# Autodesk Inventor assembly: robot
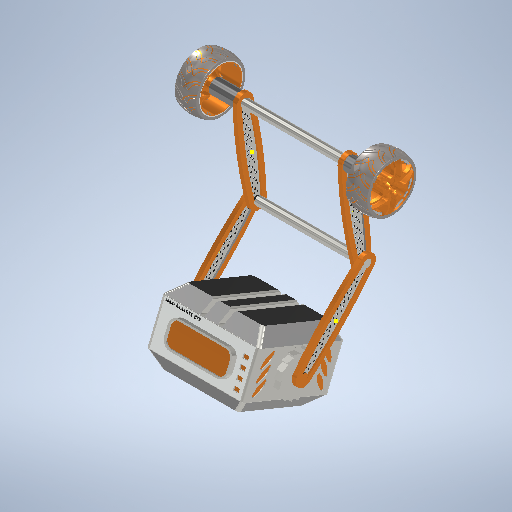
[picture p0: Inventor's stored thumbnail of the model, 512x512]
Saved by Autodesk Inventor 2025 (Build 290162000, 162)
## iProperties
Created: 2024-05-31
Part Number: robot
Document SubType Name: Assembly
Designer: bartek
Author: bartek
## Documents named in this file (6)
- C:\Users\barte\Desktop\Studia\VI semestr\Roboty mobilne\Projekt\Roboty-mobilne\robot.iam
- C:\Users\barte\Desktop\Studia\VI semestr\Roboty mobilne\Projekt\Roboty-mobilne\ipt\wheel.ipt
- C:\Users\barte\Desktop\Studia\VI semestr\Roboty mobilne\Projekt\Roboty-mobilne\ipt\engine.ipt
- C:\Users\barte\Desktop\Studia\VI semestr\Roboty mobilne\Projekt\Roboty-mobilne\ipt\link.ipt
- C:\Users\barte\Desktop\Studia\VI semestr\Roboty mobilne\Projekt\Roboty-mobilne\ipt\bolt.ipt
- C:\Users\barte\Desktop\Studia\VI semestr\Roboty mobilne\Projekt\Roboty-mobilne\ipt\body.ipt
## Components (11 placed, 5 different names)
1. wheel:1 — Rigid:1
2. wheel:2 — Rigid:2, Mate:1
3. engine:1 — Rigid:2, Mate:1, Rotational:2, Rotational:4
4. engine:2 — Rigid:1, Rotational:1, Rotational:3
5. link:1 — Rotational:2, Rotational:5, Rotational:7
6. link:2 — Rotational:1, Rotational:8, Cylindrical:3
7. bolt:1 — Rotational:3, Rotational:4
8. link:3 — Rotational:5, Cylindrical:1, Mate:2
9. bolt:2 — Rotational:7, Rotational:8
10. body:1 — Cylindrical:1, Mate:2, Cylindrical:2, Mate:3
11. link:4 — Cylindrical:2, Mate:3, Cylindrical:3
## Relationships (15: RevoluteJoint 7, Mate 3, CylindricalJoint 3, WeldJoint 2)
- Rigid:1 [WeldJoint]: wheel:1 ↔ engine:2
- Rigid:2 [WeldJoint]: wheel:2 ↔ engine:1
- Mate:1: wheel:2 ↔ engine:1
- Rotational:1 [RevoluteJoint]: engine:2 ↔ link:2
- Rotational:2 [RevoluteJoint]: engine:1 ↔ link:1
- Rotational:3 [RevoluteJoint]: engine:2 ↔ bolt:1
- Rotational:4 [RevoluteJoint]: engine:1 ↔ bolt:1
- Rotational:5 [RevoluteJoint]: link:1 ↔ link:3
- Rotational:7 [RevoluteJoint]: link:1 ↔ bolt:2
- Rotational:8 [RevoluteJoint]: link:2 ↔ bolt:2
- Cylindrical:1: link:3 ↔ body:1
- Mate:2: link:3 ↔ body:1
- Cylindrical:2: body:1 ↔ link:4
- Mate:3: body:1 ↔ link:4
- Cylindrical:3: link:2 ↔ link:4
